# Autodesk Inventor assembly: Vex Traction Wheel 4x2
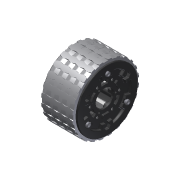
[picture p0: Inventor's stored thumbnail of the model, 180x180]
Saved by Autodesk Inventor 2013 (Build 170138000, 138)
## iProperties
Created: 2012-12-09
Part Number: Vex Traction Wheel 4x2
Document SubType Name: Assembly
Designer: Nemo
Author: Nemo
## Documents named in this file (7)
- H:\Nemo\Documents\Robotics\COTS Parts\Wheels\VexPro Traction Wheels\Vex Traction Wheel 4x2.iam
- H:\Nemo\Documents\Robotics\COTS Parts\Wheels\VexPro Traction Wheels\Components\Traction Wheel Body 4in.ipt
- H:\Nemo\Documents\Robotics\COTS Parts\Wheels\VexPro Traction Wheels\Components\Traction Wheel extension 4in.ipt
- H:\Nemo\Documents\Robotics\COTS Parts\Fasteners\8-32 locknut.ipt
- H:\Nemo\Documents\Robotics\COTS Parts\Fasteners\Hex Standoff 8-32 x1750.ipt
- H:\Nemo\Documents\Robotics\COTS Parts\Fasteners\8-32 SHCS x2250.ipt
- H:\Nemo\Documents\Robotics\COTS Parts\Wheels\VexPro Traction Wheels\Components\4 in Traction Tire.iam
## Components (20 placed, 6 different names)
1. Traction Wheel Body 4in:1 — Mate:1, Mate:2, Mate:3, Mate:4, Mate:5, Mate:6, Mate:9, Angle:1, Mate:10, Insert:2, Angle:2, Mate:14
2. Traction Wheel Body 4in:2 — Mate:3, Mate:7, Insert:1, Mate:12, Insert:4
3. Traction Wheel extension 4in:1 — Mate:4, Mate:5, Mate:6, Mate:7, Flush:1, Insert:3
4. Traction Wheel extension 4in:2 — Mate:11, Insert:3, Mate:12
5. 4 in Traction Tire:1 [sub-assembly] — Mate:13, Angle:3, Mate:14, Mate:16, Mate:17
6. 4 in Traction Tire:2 [sub-assembly] — Mate:15, Mate:16, Mate:17, Mate:19, Mate:20
7. 4 in Traction Tire:3 [sub-assembly] — Mate:18, Mate:19, Mate:20, Mate:22, Mate:23
8. 4 in Traction Tire:4 [sub-assembly] — Mate:21, Mate:22, Mate:23
9. Hex Standoff 8-32 x1750:1 — Mate:9, Angle:1, Mate:10
10. Hex Standoff 8-32 x1750:2
11. Hex Standoff 8-32 x1750:3
12. Hex Standoff 8-32 x1750:4
13. Hex Standoff 8-32 x1750:5
14. Hex Standoff 8-32 x1750:6
15. 8-32 SHCS x2250:1 — Insert:1, Insert:4
16. 8-32 locknut:1 — Insert:2, Angle:2
17. 8-32 SHCS x2250:2
18. 8-32 locknut:2
19. 8-32 SHCS x2250:3
20. 8-32 locknut:3
## Component patterns: (6 elements, first: Hex Standoff 8-32 x1750:1), (3 elements, first: 8-32 SHCS x2250:1 + 8-32 locknut:1)
## Relationships (30: Mate 22, Insert 4, Angle 3, Flush 1)
- Mate:1: Traction Wheel Body 4in:1
- Mate:2: Traction Wheel Body 4in:1
- Mate:3: Traction Wheel Body 4in:1 ↔ Traction Wheel Body 4in:2
- Mate:4: Traction Wheel Body 4in:1 ↔ Traction Wheel extension 4in:1
- Mate:5: Traction Wheel Body 4in:1 ↔ Traction Wheel extension 4in:1
- Mate:6: Traction Wheel Body 4in:1 ↔ Traction Wheel extension 4in:1
- Mate:7: Traction Wheel Body 4in:2 ↔ Traction Wheel extension 4in:1
- Mate:9: Traction Wheel Body 4in:1 ↔ Hex Standoff 8-32 x1750:1
- Angle:1 (0 deg): Traction Wheel Body 4in:1 ↔ Hex Standoff 8-32 x1750:1
- Mate:10: Traction Wheel Body 4in:1 ↔ Hex Standoff 8-32 x1750:1
- Insert:1: Traction Wheel Body 4in:2 ↔ 8-32 SHCS x2250:1
- Insert:2: Traction Wheel Body 4in:1 ↔ 8-32 locknut:1
- Angle:2 (0 deg): Traction Wheel Body 4in:1 ↔ 8-32 locknut:1
- Flush:1: Traction Wheel extension 4in:1
- Mate:11: Traction Wheel extension 4in:2
- Insert:3: Traction Wheel extension 4in:1 ↔ Traction Wheel extension 4in:2
- Mate:12: Traction Wheel Body 4in:2 ↔ Traction Wheel extension 4in:2
- Insert:4: Traction Wheel Body 4in:2 ↔ 8-32 SHCS x2250:1
- Mate:13: 4 in Traction Tire:1
- Angle:3 (15 deg): 4 in Traction Tire:1
- Mate:14: Traction Wheel Body 4in:1 ↔ 4 in Traction Tire:1
- Mate:15: 4 in Traction Tire:2
- Mate:16: 4 in Traction Tire:1 ↔ 4 in Traction Tire:2
- Mate:17: 4 in Traction Tire:1 ↔ 4 in Traction Tire:2
- Mate:18: 4 in Traction Tire:3
- Mate:19: 4 in Traction Tire:2 ↔ 4 in Traction Tire:3
- Mate:20: 4 in Traction Tire:2 ↔ 4 in Traction Tire:3
- Mate:21: 4 in Traction Tire:4
- Mate:22: 4 in Traction Tire:3 ↔ 4 in Traction Tire:4
- Mate:23: 4 in Traction Tire:3 ↔ 4 in Traction Tire:4
